# Autodesk Inventor assembly: Pickup Motor
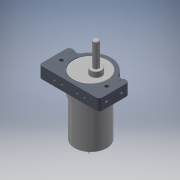
[picture p0: Inventor's stored thumbnail of the model, 180x180]
Saved by Autodesk Inventor 2016 (Build 200138000, 138)
## iProperties
Created: 2015-11-25
Part Number: Pickup Motor
Document SubType Name: Assembly
Designer: Julia
Author: Julia
## Documents named in this file (4)
- C:\Users\Aeolus\Documents\GitHub\RobotuxCAD\FTC CAD Parts\Pickup Motor.iam
- C:\Users\Aeolus\Documents\GitHub\RobotuxCAD\FTC CAD Parts\Tetrix Motor.ipt
- C:\Users\Aeolus\Documents\GitHub\RobotuxCAD\FTC CAD Parts\Tetrix Parts\tetrix_739376x108129_2013.ipt
- C:\Users\Aeolus\Documents\GitHub\RobotuxCAD\FTC CAD Parts\Tetrix Parts\tetrix_739376x108128_2013.ipt
## Components (3 placed, 3 different names)
1. Tetrix Motor:1 — Mate:1, Flush:1
2. tetrix_739376x108129_2013:1 — Mate:1, Mate:2, Mate:3, Mate:4, Flush:1
3. tetrix_739376x108128_2013:1 — Mate:2, Mate:3, Mate:4
## Relationships (5: Mate 4, Flush 1)
- Mate:1: Tetrix Motor:1 ↔ tetrix_739376x108129_2013:1
- Mate:2: tetrix_739376x108129_2013:1 ↔ tetrix_739376x108128_2013:1
- Mate:3: tetrix_739376x108129_2013:1 ↔ tetrix_739376x108128_2013:1
- Mate:4: tetrix_739376x108129_2013:1 ↔ tetrix_739376x108128_2013:1
- Flush:1: Tetrix Motor:1 ↔ tetrix_739376x108129_2013:1
